# Autodesk Inventor assembly: 下半身_6
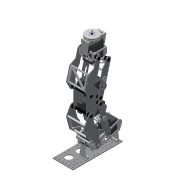
[picture p0: Inventor's stored thumbnail of the model, 180x180]
Saved by Autodesk Inventor 2016 (Build 200138000, 138)
## iProperties
Created: 2016-08-23
Part Number: 下半身_6
Material: 一般
Document SubType Name: Assembly
Designer: hiro
Mass: 908.966 g
Surface Area: 2435.97 cm^2
Volume: 423.983 cm^3
Density: 2.14387 g/cm^3
Author: hiro
## Documents named in this file (15)
- C:\Users\haya\Desktop\OpenPlatform\下半身_6_MIR.iam
- C:\Users\haya\Desktop\OpenPlatform\下半身\足首\足首_1.iam
- C:\Users\haya\Desktop\OpenPlatform\下半身\足首\足首_独立ピッチ_1.iam
- C:\Users\haya\Desktop\OpenPlatform\下半身_160823\リンク\リンク_6_1.iam
- C:\Users\haya\Desktop\OpenPlatform\下半身_160823\リンク\長穴減速_ホーン_1.iam
- C:\Users\haya\Desktop\OpenPlatform\下半身_160823\リンク\リンク_6_2.iam
- C:\Users\haya\Desktop\OpenPlatform\下半身_160823\リンク\リンク_6_3.iam
- C:\Users\haya\Desktop\OpenPlatform\下半身_160823\リンク\長穴減速_ホーン_1_MIR.iam
- C:\Users\haya\Desktop\OpenPlatform\下半身_160823\リンク\リンク_6_4.iam
- C:\Users\haya\Desktop\OpenPlatform\下半身_160823\付け根ロール\付け根ロール_6.iam
- C:\Users\haya\Desktop\OpenPlatform\下半身_160823\付け根ロール\長穴減速_ホーン_2.iam
- C:\Users\haya\Desktop\OpenPlatform\下半身_160823\リンク\長穴減速_ホーン_2.iam
- C:\Users\haya\Desktop\OpenPlatform\下半身\足裏\足裏_1_1_MIR.iam
- C:\Users\haya\Desktop\OpenPlatform\下半身_160823\膝\膝_6_1_MIR.iam
- C:\Users\haya\Desktop\OpenPlatform\下半身_160823\付け根\付け根_6_1_MIR.iam
## Components (16 placed, 13 different names)
1. 付け根ロール_6:1 [sub-assembly] — メイト:23, フラッシュ:25, フラッシュ:26, 角度:3, メイト:25, 挿入:65, 挿入:66, 角度:22, 角度:23, 角度:24
2. 足首_1:1 [sub-assembly] — 挿入:22, 挿入:23, 挿入:28, 挿入:29, 挿入:30, 挿入:31, 挿入:49, 挿入:50
3. 足首_独立ピッチ_1:1 [sub-assembly] — 挿入:22, 挿入:23, 挿入:25, 挿入:24, 挿入:26, 挿入:27, 挿入:28, 挿入:29, 挿入:30, 挿入:31
4. 長穴減速_ホーン_1:1 [sub-assembly] — 挿入:48, 挿入:63
5. 長穴減速_ホーン_1_MIR:1 [sub-assembly] — 挿入:47, 挿入:64
6. 長穴減速_ホーン_2:1 [sub-assembly] — 挿入:46, 挿入:67
7. リンク_6_3:1 [sub-assembly] — メイト:26, 挿入:53, 挿入:54, 挿入:70, 挿入:71
8. リンク_6_1:1 [sub-assembly] — 挿入:25, 挿入:24, メイト:27, 挿入:55, 挿入:57
9. リンク_6_4:1 [sub-assembly] — 角度:18, 角度:19, 角度:20, 角度:21, 挿入:51, 挿入:52, 挿入:68, 挿入:69
10. リンク_6_2:1 [sub-assembly] — 角度:14, 角度:15, 角度:16, 角度:17, 挿入:26, 挿入:27, 挿入:56, 挿入:58
11. 長穴減速_ホーン_2:2 [sub-assembly] — 挿入:46, メイト:25
12. 長穴減速_ホーン_2:3 [sub-assembly] — 挿入:48, メイト:27
13. 長穴減速_ホーン_2:4 [sub-assembly] — 挿入:47, メイト:26
14. 足裏_1_1_MIR:1 [sub-assembly] — 角度:3, 挿入:49, 挿入:50
15. 膝_6_1_MIR:1 [sub-assembly] — 角度:16, 角度:20, 角度:18, 角度:14, 角度:15, 角度:19, 角度:17, 角度:21, 挿入:51, 挿入:52, 挿入:53, 挿入:54, 挿入:55, 挿入:56, 挿入:57, 挿入:58, 挿入:63, 挿入:64
16. 付け根_6_1_MIR:1 [sub-assembly] — 挿入:65, 挿入:66, 挿入:67, 角度:22, 角度:23, 角度:24, 挿入:68, 挿入:69, 挿入:70, 挿入:71
## Relationships (50: Insert 32, Angle 12, Mate 4, Flush 2)
- 角度:3 [Angle] (0 deg): 付け根ロール_6:1 ↔ 足裏_1_1_MIR:1
- 角度:14 [Angle] (0 deg): リンク_6_2:1 ↔ 膝_6_1_MIR:1
- 角度:15 [Angle] (-30 deg): リンク_6_2:1 ↔ 膝_6_1_MIR:1
- 角度:16 [Angle] (15 deg): リンク_6_2:1 ↔ 膝_6_1_MIR:1
- 角度:17 [Angle] (90 deg): リンク_6_2:1 ↔ 膝_6_1_MIR:1
- 角度:18 [Angle] (0 deg): リンク_6_4:1 ↔ 膝_6_1_MIR:1
- 角度:19 [Angle] (30 deg): リンク_6_4:1 ↔ 膝_6_1_MIR:1
- 角度:20 [Angle] (-15 deg): リンク_6_4:1 ↔ 膝_6_1_MIR:1
- 角度:21 [Angle] (90 deg): リンク_6_4:1 ↔ 膝_6_1_MIR:1
- メイト:23 [Mate]: 付け根ロール_6:1
- フラッシュ:25 [Flush]: 付け根ロール_6:1
- フラッシュ:26 [Flush]: 付け根ロール_6:1
- 挿入:22 [Insert]: 足首_1:1 ↔ 足首_独立ピッチ_1:1
- 挿入:23 [Insert]: 足首_1:1 ↔ 足首_独立ピッチ_1:1
- 挿入:26 [Insert]: 足首_独立ピッチ_1:1 ↔ リンク_6_2:1
- 挿入:27 [Insert]: 足首_独立ピッチ_1:1 ↔ リンク_6_2:1
- 挿入:28 [Insert]: 足首_1:1 ↔ 足首_独立ピッチ_1:1
- 挿入:29 [Insert]: 足首_1:1 ↔ 足首_独立ピッチ_1:1
- 挿入:30 [Insert]: 足首_1:1 ↔ 足首_独立ピッチ_1:1
- 挿入:31 [Insert]: 足首_1:1 ↔ 足首_独立ピッチ_1:1
- 挿入:25 [Insert]: 足首_独立ピッチ_1:1 ↔ リンク_6_1:1
- 挿入:24 [Insert]: 足首_独立ピッチ_1:1 ↔ リンク_6_1:1
- 挿入:46 [Insert]: 長穴減速_ホーン_2:1 ↔ 長穴減速_ホーン_2:2
- メイト:25 [Mate]: 付け根ロール_6:1 ↔ 長穴減速_ホーン_2:2
- 挿入:47 [Insert]: 長穴減速_ホーン_1_MIR:1 ↔ 長穴減速_ホーン_2:4
- 挿入:48 [Insert]: 長穴減速_ホーン_1:1 ↔ 長穴減速_ホーン_2:3
- メイト:26 [Mate]: リンク_6_3:1 ↔ 長穴減速_ホーン_2:4
- メイト:27 [Mate]: リンク_6_1:1 ↔ 長穴減速_ホーン_2:3
- 挿入:49 [Insert]: 足首_1:1 ↔ 足裏_1_1_MIR:1
- 挿入:50 [Insert]: 足首_1:1 ↔ 足裏_1_1_MIR:1
- 挿入:51 [Insert]: リンク_6_4:1 ↔ 膝_6_1_MIR:1
- 挿入:52 [Insert]: リンク_6_4:1 ↔ 膝_6_1_MIR:1
- 挿入:53 [Insert]: リンク_6_3:1 ↔ 膝_6_1_MIR:1
- 挿入:54 [Insert]: リンク_6_3:1 ↔ 膝_6_1_MIR:1
- 挿入:55 [Insert]: リンク_6_1:1 ↔ 膝_6_1_MIR:1
- 挿入:56 [Insert]: リンク_6_2:1 ↔ 膝_6_1_MIR:1
- 挿入:57 [Insert]: リンク_6_1:1 ↔ 膝_6_1_MIR:1
- 挿入:58 [Insert]: リンク_6_2:1 ↔ 膝_6_1_MIR:1
- 挿入:63 [Insert]: 長穴減速_ホーン_1:1 ↔ 膝_6_1_MIR:1
- 挿入:64 [Insert]: 長穴減速_ホーン_1_MIR:1 ↔ 膝_6_1_MIR:1
- 挿入:65 [Insert]: 付け根ロール_6:1 ↔ 付け根_6_1_MIR:1
- 挿入:66 [Insert]: 付け根ロール_6:1 ↔ 付け根_6_1_MIR:1
- 挿入:67 [Insert]: 長穴減速_ホーン_2:1 ↔ 付け根_6_1_MIR:1
- 角度:22 [Angle] (0 deg): 付け根ロール_6:1 ↔ 付け根_6_1_MIR:1
- 角度:23 [Angle] (45 deg): 付け根ロール_6:1 ↔ 付け根_6_1_MIR:1
- 角度:24 [Angle] (20 deg): 付け根ロール_6:1 ↔ 付け根_6_1_MIR:1
- 挿入:68 [Insert]: リンク_6_4:1 ↔ 付け根_6_1_MIR:1
- 挿入:69 [Insert]: リンク_6_4:1 ↔ 付け根_6_1_MIR:1
- 挿入:70 [Insert]: リンク_6_3:1 ↔ 付け根_6_1_MIR:1
- 挿入:71 [Insert]: リンク_6_3:1 ↔ 付け根_6_1_MIR:1
## Named parameters: sa_0 = 80000, sa_1 = -5.398e-10, sa_2 = 3.965e-10
note: some values were not read from the file. Shown as the stored number, unit unknown: "sa_0", "sa_1", "sa_2".
